# Autodesk Inventor assembly: 3-finger_gripper_finger_C
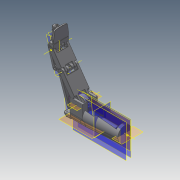
[picture p0: Inventor's stored thumbnail of the model, 180x180]
Saved by Autodesk Inventor 2018 (Build 220112000, 112)
## iProperties
Created: 2019-03-15
Part Number: 3-finger_gripper_finger_C
Document SubType Name: Assembly
Designer: Tsche
Author: Tsche
## Documents named in this file (6)
- C:\Users\Tsche\Documents\3d-printer\parts\grippers\Three_Finger_Gripper\BetaBots-Robot-Arm-Project-master\BetaBots-Robot-Arm-Project-master\ThreeFingerGripper\inventor\Gripper\3-finger_gripper_finger_C.iam
- C:\Users\Tsche\Documents\3d-printer\parts\grippers\Three_Finger_Gripper\BetaBots-Robot-Arm-Project-master\BetaBots-Robot-Arm-Project-master\ThreeFingerGripper\inventor\Gripper\finger-main_C.ipt
- C:\Users\Tsche\Documents\3d-printer\parts\grippers\Three_Finger_Gripper\BetaBots-Robot-Arm-Project-master\BetaBots-Robot-Arm-Project-master\ThreeFingerGripper\inventor\Gripper\tilt-gear_C2.ipt
- C:\Users\Tsche\Documents\3d-printer\parts\grippers\Three_Finger_Gripper\BetaBots-Robot-Arm-Project-master\BetaBots-Robot-Arm-Project-master\ThreeFingerGripper\inventor\Gripper\mirror_assembly.ipt
- C:\Users\Tsche\Documents\3d-printer\parts\grippers\Three_Finger_Gripper\BetaBots-Robot-Arm-Project-master\BetaBots-Robot-Arm-Project-master\ThreeFingerGripper\inventor\Gripper\finger_part_a.ipt
- C:\Users\Tsche\Documents\3d-printer\parts\grippers\Three_Finger_Gripper\BetaBots-Robot-Arm-Project-master\BetaBots-Robot-Arm-Project-master\ThreeFingerGripper\inventor\Gripper\finger_part_b.ipt
## Components (5 placed, 5 different names)
1. finger-main_C:1 — Mate:1, Mate:2, Mate:3, Cylindrical:1, Flush:4
2. tilt-gear_C2:1 — Mate:1, Mate:2, Mate:3
3. mirror_assembly:1 — Flush:1, Flush:2, Flush:3
4. finger_part_a:1 — Cylindrical:1, Flush:4, Cylindrical:2, Flush:5
5. finger_part_b:1 — Cylindrical:2, Flush:5
## Relationships (10: Flush 5, Mate 3, CylindricalJoint 2)
- Mate:1: finger-main_C:1 ↔ tilt-gear_C2:1
- Mate:2: finger-main_C:1 ↔ tilt-gear_C2:1
- Mate:3: finger-main_C:1 ↔ tilt-gear_C2:1
- Flush:1: mirror_assembly:1
- Flush:2: mirror_assembly:1
- Flush:3: mirror_assembly:1
- Cylindrical:1: finger-main_C:1 ↔ finger_part_a:1
- Flush:4: finger-main_C:1 ↔ finger_part_a:1
- Cylindrical:2: finger_part_a:1 ↔ finger_part_b:1
- Flush:5: finger_part_a:1 ↔ finger_part_b:1
